# Autodesk Inventor assembly: fengmingplayer
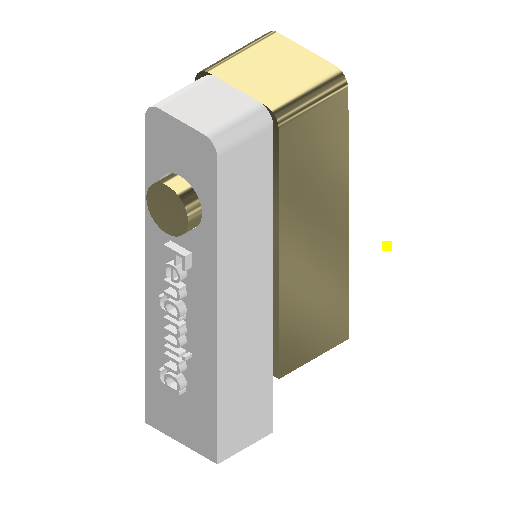
[picture p0: Inventor's stored thumbnail of the model, 512x512]
Saved by Autodesk Inventor 2025 (Build 290162000, 162)
## iProperties
Created: 2024-11-17
Part Number: fengmingplayer
Document SubType Name: Assembly
Designer: wj
Author: wj
## Documents named in this file (3)
- C:\Users\wj\Documents\fengmingplayer.iam
- C:\Users\wj\Documents\fengmingbodyplayer.ipt
- C:\Users\wj\Documents\fengmingplayerleg.ipt
## Components (2 placed, 2 different names)
1. fengmingbodyplayer:1 — Mate:1, Tangent:1
2. fengmingplayerleg:1 — Mate:1, Tangent:1
## Relationships (2: Mate 1, Tangent 1)
- Mate:1: fengmingbodyplayer:1 ↔ fengmingplayerleg:1
- Tangent:1: fengmingbodyplayer:1 ↔ fengmingplayerleg:1
